# Autodesk Inventor assembly: CB185-120
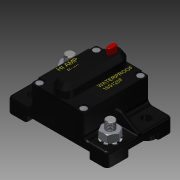
[picture p0: Inventor's stored thumbnail of the model, 180x180]
Saved by Autodesk Inventor 2014 SP1 (Build 180222100, 222)
## iProperties
Category: Electrical
Company: Autodesk Inc.
Shininess: 64.0
Length Units: 11272
Angle Units: 11279
Time Units: 11290
Mass Units: 11286
Length Display Precision: 3
Angle Display Precision: 2
Compacted: True
Part Number: CB185-120
Document SubType Name: Assembly
Created: 2012-11-26
Designer: Autodesk Inc.
Catalog Web Link: http://www.cooperindustries.com/content/dam/public/bussmann/Transportation/Circuit%20Protection/resources/datasheets/BUS_Tns_DS_18X_CIRCUITBREAKER.pdf
Description: Circuit breaker 120v
Vendor: Cooper Bussmann
Mass: 75.1287 g
Surface Area: 208.702 cm^2
Volume: 60.0434 cm^3
Density: 1.25124 g/cm^3
Density: 0.0
Volumn: 0.0
Area: 0.0
PropertySet Name: Model Information
Control State: 0
Master: False
Checked Out: False
Author: Autodesk Inc.
## Documents named in this file (8)
- C:\Users\Moses\Documents\Inventor\Sally Rebuild\Rebuild Sally\Circuit Breaker\ELEC_CircuitBreaker_CB185-120.iam
- C:\Users\Moses\Documents\Inventor\Sally Rebuild\Rebuild Sally\Circuit Breaker\BUSS-BASE.ipt
- C:\Users\Moses\Documents\Inventor\Sally Rebuild\Rebuild Sally\Circuit Breaker\BUSS-COVER.ipt
- C:\Users\Moses\Documents\Inventor\Sally Rebuild\Rebuild Sally\Circuit Breaker\BUSS-SAFTY-TRIP.ipt
- C:\Users\Moses\Documents\Inventor\Sally Rebuild\Rebuild Sally\Circuit Breaker\BUSS-RIVET.ipt
- C:\Users\Moses\Documents\Inventor\Sally Rebuild\Rebuild Sally\Circuit Breaker\BUSS-STUD-250X50.ipt
- C:\Users\Moses\Documents\Inventor\Sally Rebuild\Rebuild Sally\Circuit Breaker\ANSI B18.2.2 - 1_4 - 28(2).ipt
- C:\Users\Moses\Documents\Inventor\Sally Rebuild\Rebuild Sally\Circuit Breaker\local.ANSI.1059.80.1.ipt
## Components (13 placed, 7 different names)
1. BUSS-BASE:1 — Mate:10, Flush:1, Mate:11, Flush:2, Flush:3, Flush:4, Mate:16, Insert:1, Insert:2
2. BUSS-COVER:1 — Mate:1, Mate:2, Mate:3, Mate:4, Mate:5, Mate:6, Mate:7, Mate:8, Mate:9, Mate:10, Flush:3, Flush:4, Mate:12, Mate:13, Mate:14, Angle:1
3. BUSS-SAFTY-TRIP:1 — Mate:1, Mate:12, Mate:13, Mate:15
4. BUSS-RIVET:1 — Mate:2, Mate:3
5. BUSS-RIVET:2 — Mate:4, Mate:7
6. BUSS-RIVET:3 — Mate:5, Mate:8
7. BUSS-RIVET:4 — Mate:6, Mate:9
8. BUSS-STUD-250X50:1 — Flush:1, Mate:16
9. BUSS-STUD-250X50:2 — Mate:11, Flush:2
10. Hex Nut - Inch 1/4 - 28:1 — Insert:3
11. Hex Nut - Inch 1/4 - 28:2 — Insert:4
12. External Tooth Lock Washer - Type A (Inch) 1/4. Carbon Steel:1 — Insert:2, Insert:4
13. External Tooth Lock Washer - Type A (Inch) 1/4. Carbon Steel:2 — Insert:1, Insert:3
## Relationships (25: Mate 16, Flush 4, Insert 4, Angle 1)
- Mate:1: BUSS-COVER:1 ↔ BUSS-SAFTY-TRIP:1
- Mate:2: BUSS-COVER:1 ↔ BUSS-RIVET:1
- Mate:3: BUSS-COVER:1 ↔ BUSS-RIVET:1
- Mate:4: BUSS-COVER:1 ↔ BUSS-RIVET:2
- Mate:5: BUSS-COVER:1 ↔ BUSS-RIVET:3
- Mate:6: BUSS-COVER:1 ↔ BUSS-RIVET:4
- Mate:7: BUSS-COVER:1 ↔ BUSS-RIVET:2
- Mate:8: BUSS-COVER:1 ↔ BUSS-RIVET:3
- Mate:9: BUSS-COVER:1 ↔ BUSS-RIVET:4
- Mate:10: BUSS-BASE:1 ↔ BUSS-COVER:1
- Flush:1: BUSS-BASE:1 ↔ BUSS-STUD-250X50:1
- Mate:11: BUSS-BASE:1 ↔ BUSS-STUD-250X50:2
- Flush:2: BUSS-BASE:1 ↔ BUSS-STUD-250X50:2
- Flush:3: BUSS-BASE:1 ↔ BUSS-COVER:1
- Flush:4: BUSS-BASE:1 ↔ BUSS-COVER:1
- Mate:12: BUSS-COVER:1 ↔ BUSS-SAFTY-TRIP:1
- Mate:13: BUSS-COVER:1 ↔ BUSS-SAFTY-TRIP:1
- Mate:14: BUSS-COVER:1
- Angle:1 (0 deg): BUSS-COVER:1
- Mate:15: BUSS-SAFTY-TRIP:1
- Mate:16: BUSS-BASE:1 ↔ BUSS-STUD-250X50:1
- Insert:1: BUSS-BASE:1 ↔ External Tooth Lock Washer - Type A (Inch) 1/4. Carbon Steel:2
- Insert:2: BUSS-BASE:1 ↔ External Tooth Lock Washer - Type A (Inch) 1/4. Carbon Steel:1
- Insert:3: Hex Nut - Inch 1/4 - 28:1 ↔ External Tooth Lock Washer - Type A (Inch) 1/4. Carbon Steel:2
- Insert:4: Hex Nut - Inch 1/4 - 28:2 ↔ External Tooth Lock Washer - Type A (Inch) 1/4. Carbon Steel:1
